# Autodesk Inventor assembly: Tiger
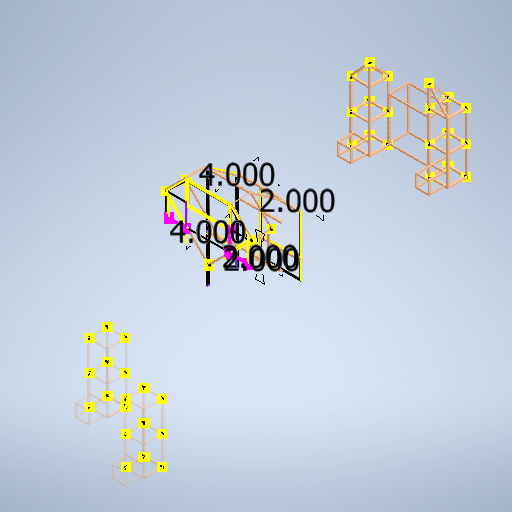
[picture p0: Inventor's stored thumbnail of the model, 512x512]
Saved by Autodesk Inventor 2025 (Build 290162000, 162)
## iProperties
Created: 2024-06-05
Part Number: Tiger
Document SubType Name: Assembly
Designer: Cupri
Mass: 180546 g
Surface Area: 136258 cm^2
Volume: 328266 cm^3
Density: 0.55 g/cm^3
Author: Cupri
## Documents named in this file (26)
- C:\Users\localadmin\Documents\USCTigerBurn24\v2\Tiger.iam
- C:\Users\localadmin\Documents\USCTigerBurn24\Standard Timber\4x4x72.ipt
- C:\Users\localadmin\Documents\USCTigerBurn24\Standard Timber\4x4x40.ipt
- C:\Users\localadmin\Documents\USCTigerBurn24\Standard Timber\2x4x36.ipt
- C:\Users\localadmin\Documents\USCTigerBurn24\Standard Timber\2x4x40.ipt
- C:\Users\localadmin\Documents\USCTigerBurn24\Standard Timber\2x4x24.ipt
- C:\Users\localadmin\Documents\USCTigerBurn24\Standard Timber\2x4x28.ipt
- C:\Users\localadmin\Documents\USCTigerBurn24\Standard Timber\2x4x72 (45 90).ipt
- C:\Users\localadmin\Documents\USCTigerBurn24\Standard Timber\2x4x68 (45 90).ipt
- C:\Users\localadmin\Documents\USCTigerBurn24\Standard Timber\2x4x42.343 (45 90).ipt
- C:\Users\localadmin\Documents\USCTigerBurn24\Standard Timber\2x4x72 (30 90).ipt
- C:\Users\localadmin\Documents\USCTigerBurn24\Standard Timber\2x4x44.ipt
- C:\Users\localadmin\Documents\USCTigerBurn24\Standard Timber\4x4x104.303.ipt
- C:\Users\localadmin\Documents\USCTigerBurn24\Standard Timber\4x4xidkanymore.ipt
- C:\Users\localadmin\Documents\USCTigerBurn24\Standard Timber\4x4x48.ipt
- C:\Users\localadmin\Documents\USCTigerBurn24\Standard Timber\4x4xigiveup.ipt
- C:\Users\localadmin\Documents\USCTigerBurn24\Standard Timber\4x4x96.ipt
- C:\Users\localadmin\Documents\USCTigerBurn24\Standard Timber\2x4x96.ipt
- C:\Users\localadmin\Documents\USCTigerBurn24\Standard Timber\2x4xidk.ipt
- C:\Users\localadmin\Documents\Back right leg.ipt
- C:\Users\localadmin\Documents\USCTigerBurn24\v2\Tiger\AIP\FEA\epzzwi8io.fins
- C:\Users\localadmin\Documents\USCTigerBurn24\v2\Tiger\AIP\FEA\epzzwi8io.fsat
- C:\Users\localadmin\Documents\USCTigerBurn24\v2\Tiger\AIP\FEA\epzzwi8io.ftes
- C:\Users\localadmin\Documents\USCTigerBurn24\v2\Tiger\AIP\FEA\epzzwi8io.fwiz
- C:\Users\localadmin\Documents\USCTigerBurn24\v2\Tiger\AIP\FEA\epzzwi8jk.fmsh
- C:\Users\localadmin\Documents\USCTigerBurn24\v2\Tiger\AIP\FEA\epzzwi8jl.fres
## Components (173 placed, 19 different names)
1. 4x4x104.303:1 — Flush:221, Flush:222
2. 4x4x104.303:2 — Flush:221, Flush:222
3. 4x4xigiveup:1 — Mate:186
4. 4x4xigiveup:2 — Flush:237, Mate:187, Mate:188
5. 4x4x96:1 — Flush:232
6. 4x4x96:2 — Flush:232
7. 4x4x96:3 — Flush:230
8. 4x4x96:4 — Flush:230
9. 4x4x96:5
10. 2x4x96:1 — Mate:186, Flush:237, Mate:187, Mate:188, Mate:191
11. 2x4xidk:1 — Mate:189, Mate:190, Mate:191, Flush:241
12. 2x4xidk:2 — Mate:192, Flush:240, Flush:241
13. Back right leg:1
14. 2x4x96:2 — Mate:260, Mate:261, Mate:262, Mate:263, Mate:264, Flush:347, Mate:286
15. 2x4x96:3 — Mate:265, Mate:266, Mate:283, Mate:284
16. 2x4x44:5 — Mate:260, Mate:261, Mate:262
17. 2x4x44:7 — Mate:263, Mate:264, Mate:265, Mate:266, Mate:285
18. 2x4x96:4 — Mate:277, Mate:278, Mate:279, Mate:280
19. 2x4x96:5 — Mate:275, Mate:281, Mate:282
20. 2x4x44:8 — Mate:274, Mate:276
21. 2x4x44:9
22. 2x4x96:8 — Mate:274, Mate:275, Mate:276, Mate:283
23. 2x4x96:9 — Mate:277, Mate:278, Flush:347, Mate:286
24. 2x4x96:10 — Mate:279, Mate:280, Mate:285, Flush:348
25. 2x4x96:11 — Mate:281, Mate:282, Mate:284, Mate:287
26. 2x4x72 (45 90):1 — Flush:88
27. 2x4x68 (45 90):1 — Flush:44, Flush:88
28. 2x4x72 (45 90):2 — Flush:48, Mate:48, Flush:51, Mate:49
29. 2x4x72 (45 90):3 — Flush:44, Mate:45, Mate:50, Flush:52, Mate:51
30. 2x4x42.343 (45 90):1 — Flush:48
31. 2x4x42.343 (45 90):2 — Mate:45
32. 2x4x72 (30 90):1 — Mate:48, Flush:51, Mate:49, Flush:70, Flush:238, Mate:192, Flush:240
33. 2x4x72 (30 90):2 — Mate:50, Flush:52, Mate:51, Flush:71, Flush:72
34. 2x4x72 (45 90):4 — Mate:61, Flush:61, Flush:62
35. 2x4x68 (45 90):2 — Mate:61, Flush:61, Flush:62
36. 2x4x72 (45 90):5 — Flush:59, Mate:59, Mate:65, Flush:67, Flush:68
37. 2x4x72 (45 90):6 — Flush:63, Flush:64, Mate:68, Flush:73
38. 2x4x42.343 (45 90):3 — Flush:59, Mate:59
39. 2x4x42.343 (45 90):4 — Flush:63
40. 2x4x72 (30 90):3 — Mate:66, Flush:69, Flush:204, Mate:189
41. 2x4x72 (30 90):4 — Flush:64, Mate:67, Mate:69, Flush:239
42. 2x4x44:1 — Mate:67, Flush:71, Flush:72, Flush:239, Mate:190
43. 2x4x44:2 — Mate:65, Flush:67, Flush:68
44. 2x4x44:3 — Mate:66, Flush:69, Flush:70, Flush:204, Flush:238
45. 2x4x44:4 — Mate:68, Flush:73, Mate:69
46. 4x4x72:49
47. 4x4x72:50 — Mate:287, Flush:348
48. 4x4x40:93
49. 4x4x40:94
50. 4x4x40:95
51. 4x4x40:96
52. 4x4x40:97
53. 4x4x40:98
54. 4x4x40:99
55. 4x4x40:100
56. 4x4x72:51
57. 4x4x72:52
58. 2x4x40:5
59. 2x4x36:17
60. 2x4x36:18
61. 2x4x36:19
62. 2x4x36:20
63. 2x4x24:9
64. 2x4x24:10
65. 2x4x28:9
66. 2x4x28:10
67. 4x4x72:53
68. 4x4x72:54
69. 4x4x40:101
70. 4x4x40:102
71. 4x4x40:103
72. 4x4x40:104
73. 4x4x72:55
74. 4x4x72:56
75. 4x4xidkanymore:5
76. 4x4x48:3
77. 4x4xidkanymore:6
78. 4x4x72:57
79. 4x4x72:58
80. 4x4x40:105
81. 4x4x40:106
82. 4x4x40:107
83. 4x4x40:108
84. 4x4x40:109
85. 4x4x40:110
86. 4x4x40:111
87. 4x4x40:112
88. 4x4x72:59
89. 4x4x72:60
90. 2x4x40:6
91. 2x4x36:21
92. 2x4x36:22
93. 2x4x36:23
94. 2x4x36:24
95. 2x4x24:11
96. 2x4x24:12
97. 2x4x28:11
98. 2x4x28:12
99. 4x4x72:61
100. 4x4x72:62
101. 4x4x40:113
102. 4x4x40:114
103. 4x4x40:115
104. 4x4x40:116
105. 4x4x72:63
106. 4x4x72:64
107. 4x4xidkanymore:7
108. 4x4x48:4
109. 4x4xidkanymore:8
110. 4x4x72:65
111. 4x4x72:66
112. 4x4x40:117
113. 4x4x40:118
114. 4x4x40:119
115. 4x4x40:120
116. 4x4x40:121
117. 4x4x40:122
118. 4x4x40:123
119. 4x4x40:124
120. 4x4x72:67
121. 4x4x72:68
122. 4x4x40:125
123. 4x4x40:126
124. 4x4x40:127
125. 2x4x40:7
126. 2x4x36:25
127. 2x4x36:26
128. 2x4x36:27
129. 2x4x36:28
130. 2x4x24:13
131. 2x4x24:14
132. 2x4x28:13
133. 2x4x28:14
134. 4x4x72:69
135. 4x4x72:70
136. 4x4x40:128
137. 4x4x40:129
138. 4x4x40:130
139. 4x4x40:131
140. 4x4x72:71
141. 4x4x72:72
142. 4x4x72:73
143. 4x4x72:74
144. 4x4x40:132
145. 4x4x40:133
146. 4x4x40:134
147. 4x4x40:135
148. 4x4x40:136
149. 4x4x40:137
150. 4x4x40:138
151. 4x4x40:139
152. 4x4x72:75
153. 4x4x72:76
154. 4x4x40:140
155. 4x4x40:141
156. 4x4x40:142
157. 2x4x40:8
158. 2x4x36:29
159. 2x4x36:30
160. 2x4x36:31
161. 2x4x36:32
162. 2x4x24:15
163. 2x4x24:16
164. 2x4x28:15
165. 2x4x28:16
166. 4x4x72:77
167. 4x4x72:78
168. 4x4x40:143
169. 4x4x40:144
170. 4x4x40:145
171. 4x4x40:146
172. 4x4x72:79
173. 4x4x72:80
## Relationships (335: Flush 138, Mate 119, WeldJoint 78)
- Flush:44: 2x4x68 (45 90):1 ↔ 2x4x72 (45 90):3
- Flush:48: 2x4x72 (45 90):2 ↔ 2x4x42.343 (45 90):1
- Mate:45: 2x4x72 (45 90):3 ↔ 2x4x42.343 (45 90):2
- Mate:48: 2x4x72 (45 90):2 ↔ 2x4x72 (30 90):1
- Flush:51: 2x4x72 (45 90):2 ↔ 2x4x72 (30 90):1
- Mate:49: 2x4x72 (45 90):2 ↔ 2x4x72 (30 90):1
- Mate:50: 2x4x72 (45 90):3 ↔ 2x4x72 (30 90):2
- Flush:52: 2x4x72 (45 90):3 ↔ 2x4x72 (30 90):2
- Mate:51: 2x4x72 (45 90):3 ↔ 2x4x72 (30 90):2
- [Flush]: 2x4x68 (45 90):2 ↔ 2x4x72 (45 90):6
- [Flush]: 2x4x72 (45 90):5 ↔ 2x4x42.343 (45 90):3
- [Mate]: 2x4x72 (45 90):6 ↔ 2x4x42.343 (45 90):4
- [Mate]: 2x4x72 (45 90):5 ↔ 2x4x72 (30 90):3
- [Flush]: 2x4x72 (45 90):5 ↔ 2x4x72 (30 90):3
- [Mate]: 2x4x72 (45 90):5 ↔ 2x4x72 (30 90):3
- [Mate]: 2x4x72 (45 90):6 ↔ 2x4x72 (30 90):4
- [Flush]: 2x4x72 (45 90):6 ↔ 2x4x72 (30 90):4
- [Mate]: 2x4x72 (45 90):6 ↔ 2x4x72 (30 90):4
- Flush:59: 2x4x72 (45 90):5 ↔ 2x4x42.343 (45 90):3
- Mate:59: 2x4x72 (45 90):5 ↔ 2x4x42.343 (45 90):3
- Mate:61: 2x4x72 (45 90):4 ↔ 2x4x68 (45 90):2
- Flush:61: 2x4x72 (45 90):4 ↔ 2x4x68 (45 90):2
- Flush:62: 2x4x72 (45 90):4 ↔ 2x4x68 (45 90):2
- Flush:63: 2x4x72 (45 90):6 ↔ 2x4x42.343 (45 90):4
- Flush:64: 2x4x72 (45 90):6 ↔ 2x4x72 (30 90):4
- Mate:65: 2x4x72 (45 90):5 ↔ 2x4x44:2
- Flush:67: 2x4x72 (45 90):5 ↔ 2x4x44:2
- Flush:68: 2x4x72 (45 90):5 ↔ 2x4x44:2
- Mate:66: 2x4x72 (30 90):3 ↔ 2x4x44:3
- Flush:69: 2x4x72 (30 90):3 ↔ 2x4x44:3
- Flush:70: 2x4x72 (30 90):1 ↔ 2x4x44:3
- Mate:67: 2x4x72 (30 90):4 ↔ 2x4x44:1
- Flush:71: 2x4x72 (30 90):2 ↔ 2x4x44:1
- Flush:72: 2x4x72 (30 90):2 ↔ 2x4x44:1
- Mate:68: 2x4x72 (45 90):6 ↔ 2x4x44:4
- Flush:73: 2x4x72 (45 90):6 ↔ 2x4x44:4
- Mate:69: 2x4x72 (30 90):4 ↔ 2x4x44:4
- Flush:88: 2x4x72 (45 90):1 ↔ 2x4x68 (45 90):1
- Flush:204: 2x4x72 (30 90):3 ↔ 2x4x44:3
- Flush:221: 4x4x104.303:1 ↔ 4x4x104.303:2
- Flush:222: 4x4x104.303:1 ↔ 4x4x104.303:2
- Flush:230: 4x4x96:3 ↔ 4x4x96:4
- Flush:232: 4x4x96:1 ↔ 4x4x96:2
- Mate:186: 4x4xigiveup:1 ↔ 2x4x96:1
- Flush:237: 4x4xigiveup:2 ↔ 2x4x96:1
- Mate:187: 4x4xigiveup:2 ↔ 2x4x96:1
- Mate:188: 4x4xigiveup:2 ↔ 2x4x96:1
- Flush:238: 2x4x72 (30 90):1 ↔ 2x4x44:3
- Flush:239: 2x4x72 (30 90):4 ↔ 2x4x44:1
- Mate:189: 2x4xidk:1 ↔ 2x4x72 (30 90):3
- Mate:190: 2x4xidk:1 ↔ 2x4x44:1
- Mate:191: 2x4x96:1 ↔ 2x4xidk:1
- Mate:192: 2x4xidk:2 ↔ 2x4x72 (30 90):1
- Flush:240: 2x4xidk:2 ↔ 2x4x72 (30 90):1
- Flush:241: 2x4xidk:1 ↔ 2x4xidk:2
- [WeldJoint]: 4x4x72:49 ↔ 4x4x40:93
- [WeldJoint]: 4x4x72:50 ↔ 4x4x40:93
- [WeldJoint]: 4x4x72:49 ↔ 4x4x40:94
- [WeldJoint]: 4x4x72:50 ↔ 4x4x40:96
- [WeldJoint]: 4x4x40:94 ↔ 4x4x72:51
- [WeldJoint]: 4x4x40:95 ↔ 4x4x72:51
- [WeldJoint]: 4x4x40:96 ↔ 4x4x72:52
- [WeldJoint]: 4x4x72:50 ↔ 4x4x40:97
- [WeldJoint]: 4x4x40:98 ↔ 4x4x72:51
- [WeldJoint]: 4x4x72:49 ↔ 4x4x40:100
- [WeldJoint]: 4x4x72:49 ↔ 4x4x40:99
- [Mate]: 4x4x72:51 ↔ 2x4x40:5
- [Flush]: 4x4x72:51 ↔ 2x4x40:5
- [Mate] (609.6 mm): 4x4x40:95 ↔ 2x4x40:5
- [Mate] (101.6 mm): 4x4x40:95 ↔ 2x4x36:17
- [Flush]: 4x4x40:95 ↔ 2x4x36:17
- [Mate] (101.6 mm): 4x4x72:52 ↔ 2x4x36:20
- [Flush]: 4x4x40:95 ↔ 2x4x36:20
- [Mate] (101.6 mm): 2x4x40:5 ↔ 2x4x36:18
- [Flush]: 2x4x40:5 ↔ 2x4x36:18
- [Mate]: 2x4x40:5 ↔ 2x4x36:19
- [Flush]: 2x4x40:5 ↔ 2x4x36:19
- [Mate]: 2x4x36:19 ↔ 2x4x36:20
- [WeldJoint]: 2x4x36:17 ↔ 2x4x24:9
- [WeldJoint]: 2x4x36:20 ↔ 2x4x24:10
- [WeldJoint]: 2x4x36:19 ↔ 2x4x28:9
- [WeldJoint]: 2x4x36:20 ↔ 2x4x28:10
- [WeldJoint]: 4x4x72:54 ↔ 4x4x40:101
- [WeldJoint]: 4x4x40:102 ↔ 4x4x72:55
- [WeldJoint]: 4x4x72:53 ↔ 4x4x40:104
- [WeldJoint]: 4x4x72:53 ↔ 4x4x40:103
- [Flush]: 2x4x40:5 ↔ 2x4x36:18
- [Flush]: 2x4x40:5 ↔ 2x4x36:19
- [Flush]: 4x4x40:95 ↔ 2x4x36:17
- [Flush]: 4x4x40:95 ↔ 2x4x36:20
- [Flush] (203.2 mm): 4x4x72:52 ↔ 2x4x36:19
- [Flush] (203.2 mm): 4x4x72:52 ↔ 2x4x36:20
- [Flush]: 2x4x36:17 ↔ 2x4x28:10
- [Mate]: 2x4x36:18 ↔ 2x4x28:9
- [Flush]: 4x4x40:102 ↔ 4x4x72:55
- [Flush]: 4x4x40:102 ↔ 4x4x72:56
- [Mate]: 4x4x40:102 ↔ 4x4x72:56
- [Mate]: 4x4x40:101 ↔ 4x4x72:56
- [Flush]: 4x4x40:101 ↔ 4x4x72:56
- [Flush]: 4x4x72:54 ↔ 4x4x40:101
- [Mate]: 4x4x72:54 ↔ 4x4x40:101
- [Flush]: 4x4x72:53 ↔ 4x4x40:104
- [Flush]: 4x4x72:53 ↔ 4x4x40:103
- [Mate]: 4x4x72:51 ↔ 2x4x40:5
- [Mate]: 2x4x36:18 ↔ 2x4x24:9
- [Flush]: 4x4x72:52 ↔ 4x4x72:56
- [Flush]: 4x4x72:50 ↔ 4x4x40:97
- [Mate]: 4x4x72:50 ↔ 4x4x72:54
- [Flush]: 4x4x72:50 ↔ 4x4x72:54
- [Flush]: 4x4x72:49 ↔ 4x4x72:53
- [Mate]: 4x4x72:49 ↔ 4x4x72:53
- [Flush]: 4x4x72:49 ↔ 4x4x72:53
- [Mate]: 4x4x72:51 ↔ 4x4x72:55
- [Flush]: 4x4x72:51 ↔ 4x4x72:55
- [Flush]: 4x4x72:51 ↔ 4x4x72:55
- [Mate]: 2x4x36:17 ↔ 2x4x28:10
- [Flush]: 2x4x36:18 ↔ 2x4x24:9
- [Flush]: 2x4x36:18 ↔ 2x4x28:9
- [Flush]: 4x4x72:54 ↔ 4x4x40:103
- [Flush]: 4x4x40:101 ↔ 4x4x40:104
- [Flush]: 4x4x72:53 ↔ 4x4x40:103
- [Flush]: 4x4x40:102 ↔ 4x4x72:55
- [Flush]: 4x4x40:102 ↔ 4x4x72:56
- [WeldJoint]: 4x4x72:54 ↔ 4x4xidkanymore:5
- [Flush]: 4x4x72:54 ↔ 4x4xidkanymore:5
- [Flush]: 4x4x40:101 ↔ 4x4xidkanymore:5
- [Mate]: 4x4x72:56 ↔ 4x4x48:3
- [Flush]: 4x4x72:56 ↔ 4x4x48:3
- [Flush]: 4x4x72:56 ↔ 4x4x48:3
- [Mate]: 4x4x48:3 ↔ 4x4xidkanymore:6
- [Flush]: 4x4x48:3 ↔ 4x4xidkanymore:6
- [Mate]: 4x4x40:102 ↔ 4x4xidkanymore:6
- [WeldJoint]: 4x4x72:57 ↔ 4x4x40:105
- [WeldJoint]: 4x4x72:58 ↔ 4x4x40:105
- [WeldJoint]: 4x4x72:57 ↔ 4x4x40:106
- [WeldJoint]: 4x4x72:58 ↔ 4x4x40:108
- [WeldJoint]: 4x4x40:106 ↔ 4x4x72:59
- [WeldJoint]: 4x4x40:107 ↔ 4x4x72:59
- [WeldJoint]: 4x4x40:108 ↔ 4x4x72:60
- [WeldJoint]: 4x4x72:58 ↔ 4x4x40:109
- [WeldJoint]: 4x4x40:110 ↔ 4x4x72:59
- [WeldJoint]: 4x4x72:57 ↔ 4x4x40:112
- [WeldJoint]: 4x4x72:57 ↔ 4x4x40:111
- [Mate]: 4x4x72:59 ↔ 2x4x40:6
- [Flush]: 4x4x72:59 ↔ 2x4x40:6
- [Mate] (609.6 mm): 4x4x40:107 ↔ 2x4x40:6
- [Mate] (101.6 mm): 4x4x40:107 ↔ 2x4x36:21
- [Flush]: 4x4x40:107 ↔ 2x4x36:21
- [Mate] (101.6 mm): 4x4x72:60 ↔ 2x4x36:24
- [Flush]: 4x4x40:107 ↔ 2x4x36:24
- [Mate] (101.6 mm): 2x4x40:6 ↔ 2x4x36:22
- [Flush]: 2x4x40:6 ↔ 2x4x36:22
- [Mate]: 2x4x40:6 ↔ 2x4x36:23
- [Flush]: 2x4x40:6 ↔ 2x4x36:23
- [Mate]: 2x4x36:23 ↔ 2x4x36:24
- [WeldJoint]: 2x4x36:21 ↔ 2x4x24:11
- [WeldJoint]: 2x4x36:24 ↔ 2x4x24:12
- [WeldJoint]: 2x4x36:23 ↔ 2x4x28:11
- [WeldJoint]: 2x4x36:24 ↔ 2x4x28:12
- [WeldJoint]: 4x4x72:62 ↔ 4x4x40:113
- [WeldJoint]: 4x4x40:114 ↔ 4x4x72:63
- [WeldJoint]: 4x4x72:61 ↔ 4x4x40:116
- [WeldJoint]: 4x4x72:61 ↔ 4x4x40:115
- [Flush]: 2x4x40:6 ↔ 2x4x36:22
- [Flush]: 2x4x40:6 ↔ 2x4x36:23
- [Flush]: 4x4x40:107 ↔ 2x4x36:21
- [Flush]: 4x4x40:107 ↔ 2x4x36:24
- [Flush] (203.2 mm): 4x4x72:60 ↔ 2x4x36:23
- [Flush] (203.2 mm): 4x4x72:60 ↔ 2x4x36:24
- [Flush]: 2x4x36:21 ↔ 2x4x28:12
- [Mate]: 2x4x36:22 ↔ 2x4x28:11
- [Flush]: 4x4x40:114 ↔ 4x4x72:63
- [Flush]: 4x4x40:114 ↔ 4x4x72:64
- [Mate]: 4x4x40:114 ↔ 4x4x72:64
- [Mate]: 4x4x40:113 ↔ 4x4x72:64
- [Flush]: 4x4x40:113 ↔ 4x4x72:64
- [Flush]: 4x4x72:62 ↔ 4x4x40:113
- [Mate]: 4x4x72:62 ↔ 4x4x40:113
- [Flush]: 4x4x72:61 ↔ 4x4x40:116
- [Flush]: 4x4x72:61 ↔ 4x4x40:115
- [Mate]: 4x4x72:59 ↔ 2x4x40:6
- [Mate]: 2x4x36:22 ↔ 2x4x24:11
- [Flush]: 4x4x72:60 ↔ 4x4x72:64
- [Flush]: 4x4x72:58 ↔ 4x4x40:109
- [Mate]: 4x4x72:58 ↔ 4x4x72:62
- [Flush]: 4x4x72:58 ↔ 4x4x72:62
- [Flush]: 4x4x72:57 ↔ 4x4x72:61
- [Mate]: 4x4x72:57 ↔ 4x4x72:61
- [Flush]: 4x4x72:57 ↔ 4x4x72:61
- [Mate]: 4x4x72:59 ↔ 4x4x72:63
- [Flush]: 4x4x72:59 ↔ 4x4x72:63
- [Flush]: 4x4x72:59 ↔ 4x4x72:63
- [Mate]: 2x4x36:21 ↔ 2x4x28:12
- [Flush]: 2x4x36:22 ↔ 2x4x24:11
- [Flush]: 2x4x36:22 ↔ 2x4x28:11
- [WeldJoint]: 4x4x72:61 ↔ 4x4xidkanymore:7
- [Flush]: 4x4x72:61 ↔ 4x4xidkanymore:7
- [Mate]: 4x4x72:63 ↔ 4x4x48:4
- [Flush]: 4x4x72:63 ↔ 4x4x48:4
- [Flush]: 4x4x72:63 ↔ 4x4x48:4
- [Mate]: 4x4x72:64 ↔ 4x4xidkanymore:8
- [Mate]: 4x4x48:4 ↔ 4x4xidkanymore:8
- [Flush]: 4x4x48:4 ↔ 4x4xidkanymore:8
- [WeldJoint]: 4x4x72:65 ↔ 4x4x40:117
- [WeldJoint]: 4x4x72:66 ↔ 4x4x40:117
- [WeldJoint]: 4x4x72:65 ↔ 4x4x40:118
- [WeldJoint]: 4x4x72:66 ↔ 4x4x40:120
- [WeldJoint]: 4x4x40:118 ↔ 4x4x72:67
- [WeldJoint]: 4x4x40:119 ↔ 4x4x72:67
- [WeldJoint]: 4x4x40:120 ↔ 4x4x72:68
- [WeldJoint]: 4x4x72:66 ↔ 4x4x40:121
- [WeldJoint]: 4x4x40:122 ↔ 4x4x72:67
- [WeldJoint]: 4x4x72:65 ↔ 4x4x40:124
- [WeldJoint]: 4x4x72:65 ↔ 4x4x40:123
- [Mate]: 4x4x72:67 ↔ 2x4x40:7
- [Flush]: 4x4x72:67 ↔ 2x4x40:7
- [Mate] (609.6 mm): 4x4x40:119 ↔ 2x4x40:7
- [Mate] (101.6 mm): 4x4x40:119 ↔ 2x4x36:25
- [Flush]: 4x4x40:119 ↔ 2x4x36:25
- [Mate] (101.6 mm): 4x4x72:68 ↔ 2x4x36:28
- [Flush]: 4x4x40:119 ↔ 2x4x36:28
- [Mate] (101.6 mm): 2x4x40:7 ↔ 2x4x36:26
- [Flush]: 2x4x40:7 ↔ 2x4x36:26
- [Mate]: 2x4x40:7 ↔ 2x4x36:27
- [Flush]: 2x4x40:7 ↔ 2x4x36:27
- [Mate]: 2x4x36:27 ↔ 2x4x36:28
- [WeldJoint]: 2x4x36:25 ↔ 2x4x24:13
- [WeldJoint]: 2x4x36:28 ↔ 2x4x24:14
- [WeldJoint]: 2x4x36:27 ↔ 2x4x28:13
- [WeldJoint]: 2x4x36:28 ↔ 2x4x28:14
- [WeldJoint]: 4x4x72:70 ↔ 4x4x40:128
- [WeldJoint]: 4x4x40:129 ↔ 4x4x72:71
- [WeldJoint]: 4x4x72:69 ↔ 4x4x40:131
- [WeldJoint]: 4x4x72:69 ↔ 4x4x40:130
- [Flush]: 2x4x40:7 ↔ 2x4x36:26
- [Flush]: 2x4x40:7 ↔ 2x4x36:27
- [Flush]: 4x4x40:119 ↔ 2x4x36:25
- [Flush]: 4x4x40:119 ↔ 2x4x36:28
- [Flush] (203.2 mm): 4x4x72:68 ↔ 2x4x36:27
- [Flush] (203.2 mm): 4x4x72:68 ↔ 2x4x36:28
- [Flush]: 2x4x36:25 ↔ 2x4x28:14
- [Mate]: 2x4x36:26 ↔ 2x4x28:13
- [Flush]: 4x4x40:129 ↔ 4x4x72:71
- [Flush]: 4x4x40:129 ↔ 4x4x72:72
- [Mate]: 4x4x40:129 ↔ 4x4x72:72
- [Mate]: 4x4x40:128 ↔ 4x4x72:72
- [Flush]: 4x4x40:128 ↔ 4x4x72:72
- [Flush]: 4x4x72:70 ↔ 4x4x40:128
- [Mate]: 4x4x72:70 ↔ 4x4x40:128
- [Flush]: 4x4x72:69 ↔ 4x4x40:131
- [Flush]: 4x4x72:69 ↔ 4x4x40:130
- [Mate]: 4x4x72:67 ↔ 2x4x40:7
- [Mate]: 2x4x36:26 ↔ 2x4x24:13
- [Flush]: 4x4x72:68 ↔ 4x4x72:72
- [Flush]: 4x4x72:68 ↔ 4x4x72:72
- [WeldJoint]: 4x4x72:73 ↔ 4x4x40:132
- [WeldJoint]: 4x4x72:74 ↔ 4x4x40:132
- [WeldJoint]: 4x4x72:73 ↔ 4x4x40:133
- [WeldJoint]: 4x4x72:74 ↔ 4x4x40:135
- [WeldJoint]: 4x4x40:133 ↔ 4x4x72:75
- [WeldJoint]: 4x4x40:134 ↔ 4x4x72:75
- [WeldJoint]: 4x4x40:135 ↔ 4x4x72:76
- [WeldJoint]: 4x4x72:74 ↔ 4x4x40:136
- [WeldJoint]: 4x4x40:137 ↔ 4x4x72:75
- [WeldJoint]: 4x4x72:73 ↔ 4x4x40:139
- [WeldJoint]: 4x4x72:73 ↔ 4x4x40:138
- [Mate]: 4x4x72:75 ↔ 2x4x40:8
- [Flush]: 4x4x72:75 ↔ 2x4x40:8
- [Mate] (609.6 mm): 4x4x40:134 ↔ 2x4x40:8
- [Mate] (101.6 mm): 4x4x40:134 ↔ 2x4x36:29
- [Flush]: 4x4x40:134 ↔ 2x4x36:29
- [Mate] (101.6 mm): 4x4x72:76 ↔ 2x4x36:32
- [Flush]: 4x4x40:134 ↔ 2x4x36:32
- [Mate]: 2x4x40:8 ↔ 2x4x36:31
- [Flush]: 2x4x40:8 ↔ 2x4x36:31
- [Mate]: 2x4x36:31 ↔ 2x4x36:32
- [WeldJoint]: 2x4x36:29 ↔ 2x4x24:15
- [WeldJoint]: 2x4x36:32 ↔ 2x4x24:16
- [WeldJoint]: 2x4x36:31 ↔ 2x4x28:15
- [WeldJoint]: 2x4x36:32 ↔ 2x4x28:16
- [WeldJoint]: 4x4x72:78 ↔ 4x4x40:143
- [WeldJoint]: 4x4x40:144 ↔ 4x4x72:79
- [WeldJoint]: 4x4x72:77 ↔ 4x4x40:146
- [WeldJoint]: 4x4x72:77 ↔ 4x4x40:145
- [Flush]: 2x4x40:8 ↔ 2x4x36:31
- [Flush]: 4x4x40:134 ↔ 2x4x36:29
- [Flush]: 4x4x40:134 ↔ 2x4x36:32
- [Flush] (203.2 mm): 4x4x72:76 ↔ 2x4x36:31
- [Flush] (203.2 mm): 4x4x72:76 ↔ 2x4x36:32
- [Flush]: 2x4x36:29 ↔ 2x4x28:16
- [Flush]: 2x4x36:30 ↔ 2x4x28:15
- [Mate]: 2x4x36:30 ↔ 2x4x28:15
- [Flush]: 4x4x40:144 ↔ 4x4x72:79
- [Flush]: 4x4x40:144 ↔ 4x4x72:80
- [Mate]: 4x4x40:144 ↔ 4x4x72:79
- [Mate]: 4x4x40:146 ↔ 4x4x72:79
- [Mate]: 4x4x72:74 ↔ 4x4x72:78
- [Mate]: 4x4x72:75 ↔ 2x4x40:8
- [Mate]: 2x4x40:8 ↔ 2x4x24:15
- [Flush]: 2x4x36:31 ↔ 2x4x24:16
- [Flush]: 2x4x36:31 ↔ 2x4x24:16
- [Mate]: 2x4x40:8 ↔ 2x4x36:30
- [Flush]: 2x4x36:30 ↔ 2x4x28:15
- [Flush]: 2x4x36:30 ↔ 2x4x28:15
- [Mate]: 4x4x72:78 ↔ 4x4x40:145
- Mate:260: 2x4x96:2 ↔ 2x4x44:5
- Mate:261: 2x4x96:2 ↔ 2x4x44:5
- Mate:262: 2x4x96:2 ↔ 2x4x44:5
- Mate:263: 2x4x96:2 ↔ 2x4x44:7
- Mate:264: 2x4x96:2 ↔ 2x4x44:7
- Mate:265: 2x4x96:3 ↔ 2x4x44:7
- Mate:266: 2x4x96:3 ↔ 2x4x44:7
- [Mate]: 2x4x96:4 ↔ 2x4x44:8
- [Mate]: 2x4x96:4 ↔ 2x4x44:8
- [Mate]: 2x4x96:4 ↔ 2x4x44:8
- [Mate]: 2x4x96:4 ↔ 2x4x44:9
- [Mate]: 2x4x96:4 ↔ 2x4x44:9
- [Mate]: 2x4x96:5 ↔ 2x4x44:9
- [Mate]: 2x4x96:5 ↔ 2x4x44:9
- Mate:274: 2x4x44:8 ↔ 2x4x96:8
- Mate:275: 2x4x96:5 ↔ 2x4x96:8
- Mate:276: 2x4x44:8 ↔ 2x4x96:8
- Mate:277: 2x4x96:4 ↔ 2x4x96:9
- Mate:278: 2x4x96:4 ↔ 2x4x96:9
- Mate:279: 2x4x96:4 ↔ 2x4x96:10
- Mate:280: 2x4x96:4 ↔ 2x4x96:10
- Mate:281: 2x4x96:5 ↔ 2x4x96:11
- Mate:282: 2x4x96:5 ↔ 2x4x96:11
- Mate:283: 2x4x96:3 ↔ 2x4x96:8
- Flush:347: 2x4x96:2 ↔ 2x4x96:9
- Mate:284: 2x4x96:3 ↔ 2x4x96:11
- Mate:285: 2x4x44:7 ↔ 2x4x96:10
- Mate:286: 2x4x96:2 ↔ 2x4x96:9
- Mate:287: 2x4x96:11 ↔ 4x4x72:50
- Flush:348: 2x4x96:10 ↔ 4x4x72:50
## Named parameters: sa_0 = 22241.1, d253_d234 = 0 mm, d254_d240 = 0 mm, d255_d242 = 0 mm, d256_d247 = 0 mm, d257_d248 = 0 mm, d258_d249 = 0 mm, d259_d250 = 0 mm, d260_d251 = 0 mm, d261_d252 = 0 mm, sa_1 = 980.999, d679_d599 = 0 mm, d680_d600 = 0 mm, d681_d601 = 0 mm, d682_d602 = 0 mm, d683_d603 = 0 mm, d684_d605 = 0 mm, d685_d608 = 0 mm, d686_d609 = 0 mm, d687_d610 = 0 mm, d688_d611 = 0 mm, d689_d612 = 0 mm, d690_d619 = 0 mm, d691_d620 = 0 mm, d692_d621 = 0 mm, d693_d561_d429_d35 = 0 mm, d694_d562_d430_d36 = 0 mm, d695_d563_d431_d37 = 0 mm, d696_d564_d432_d38 = 0 mm, d697_d565_d505 = 0 mm, d698_d566_d506 = 0 mm, d699_d567_d507 = 0 mm, d700_d568_d508 = 0 mm, d701_d569_d509 = 0 mm, d702_d570_d512 = 0 mm, d703_d571_d513 = 0 mm, d704_d572_d514 = 0 mm, d705_d573_d498 = 0 mm, d706_d574_d501 = 0 mm, d707_d575_d502 = 0 mm, d708_d576_d503 = 0 mm, d709_d577_d504 = 0 mm, d710_d515_d433_d39 = 0 mm, d711_d516_d434_d29 = 0 mm, d712_d517_d435_d30 = 0 mm, d713_d518_d436_d326 = 0 mm, d714_d519_d437_d327 = 0 mm, d715_d520_d438_d314 = 0 mm, d716_d521_d439_d315 = 0 mm, d717_d522_d440_d316 = 0 mm, d718_d523_d441_d317 = 0 mm, d719_d524_d442_d305 = 0 mm, d720_d525_d443_d306 = 0 mm, d721_d526_d444_d311 = 0 mm, d722_d527_d445_d312 = 0 mm, d723_d528_d446_d313 = 0 mm, d724_d529_d396_d137_d48_d37 = 0 mm, d725_d530_d397_d138_d49_d38 = 0 mm, d726_d531_d398_d139_d50_d39 = 0 mm, d727_d532_d399_d143 = 0 mm, d728_d533_d400_d144 = 0 mm, d729_d534_d401_d145 = 0 mm, d730_d535_d402_d146 = 0 mm, d731_d536_d403_d147 = 203.2 mm, d732_d537_d404_d148 = 203.2 mm, d733_d538_d405_d149 = 0 mm, d734_d539_d406_d150 = 0 mm, d735_d540_d407_d61 = 0 mm, d736_d541_d408_d62 = 0 mm, d737_d542_d409_d63 = 609.6 mm, d738_d543_d410_d68 = 101.6 mm, d739_d544_d411_d69 = 0 mm, d740_d545_d412_d70 = 101.6 mm, d741_d546_d413_d71 = 0 mm, d742_d547_d414_d72 = 101.6 mm, d743_d548_d415_d73 = 0 mm, d744_d549_d416_d74 = 0 mm, d745_d550_d417_d75 = 0 mm, d746_d551_d418_d76 = 0 mm, d747_d552_d419_d77 = 0 mm, d748_d553_d420_d78 = 0 mm, d749_d554_d421_d79 = 0 mm, d750_d555_d422_d80 = 0 mm, d751_d556_d423_d136_d47_d36 = 0 mm, d752_d557_d425_d31 = 0 mm, d753_d558_d426_d32 = 0 mm, d754_d559_d427_d33 = 0 mm, d755_d560_d428_d34 = 0 mm, d756_d606 = 0 mm, d757_d607 = 0 mm, d758_d613 = 0 mm, d759_d614 = 0 mm, d760_d615 = 0 mm, d761_d616 = 0 mm, d762_d617 = 0 mm, d763_d618 = 0 mm, d764_d502 = 0 mm, d765_d503 = 0 mm, d766_d504 = 0 mm, d767_d505 = 0 mm, d768_d506 = 0 mm, d769_d507 = 0 mm, d770_d508 = 0 mm, d771_d509 = 0 mm, d772_d512 = 0 mm, d773_d513 = 0 mm, d774_d514 = 0 mm, d775_d434_d29 = 0 mm, d776_d435_d30 = 0 mm, d777_d436_d326 = 0 mm, d778_d437_d327 = 0 mm, d779_d438_d314 = 0 mm, d780_d439_d315 = 0 mm, d781_d440_d316 = 0 mm, d782_d441_d317 = 0 mm, d783_d442_d305 = 0 mm, d784_d443_d306 = 0 mm, d785_d444_d311 = 0 mm, d786_d445_d312 = 0 mm, d787_d446_d313 = 0 mm, d788_d498 = 0 mm, d789_d501 = 0 mm, d790_d396_d137_d48_d37 = 0 mm, d791_d397_d138_d49_d38 = 0 mm, d792_d398_d139_d50_d39 = 0 mm, d793_d399_d143 = 0 mm, d794_d400_d144 = 0 mm, d795_d401_d145 = 0 mm, d796_d402_d146 = 0 mm, d797_d403_d147 = 203.2 mm, d798_d404_d148 = 203.2 mm, d799_d405_d149 = 0 mm, d800_d406_d150 = 0 mm, d801_d407_d61 = 0 mm, d802_d408_d62 = 0 mm, d803_d409_d63 = 609.6 mm, d804_d410_d68 = 101.6 mm, d805_d411_d69 = 0 mm, d806_d412_d70 = 101.6 mm, d807_d413_d71 = 0 mm, d808_d414_d72 = 101.6 mm, d809_d415_d73 = 0 mm, d810_d416_d74 = 0 mm, d811_d417_d75 = 0 mm, d812_d418_d76 = 0 mm, d813_d419_d77 = 0 mm, d814_d420_d78 = 0 mm, d815_d421_d79 = 0 mm, d816_d422_d80 = 0 mm, d817_d423_d136_d47_d36 = 0 mm, d818_d425_d31 = 0 mm, d819_d426_d32 = 0 mm, d820_d427_d33 = 0 mm, d821_d428_d34 = 0 mm, d822_d429_d35 = 0 mm, d823_d430_d36 = 0 mm, d824_d431_d37 = 0 mm, d825_d432_d38 = 0 mm, d826_d433_d39 = 0 mm, d827_d499 = 0 mm, d828_d500 = 0 mm, d829_d326 = 0 mm, d830_d327 = 0 mm, d831_d305 = 0 mm, d832_d306 = 0 mm, d833_d311 = 0 mm, d834_d312 = 0 mm, d835_d313 = 0 mm, d836_d314 = 0 mm, d837_d315 = 0 mm, d838_d316 = 0 mm, d839_d317 = 0 mm, d840_d143 = 0 mm, d841_d144 = 0 mm, d842_d145 = 0 mm, d843_d146 = 0 mm, d844_d147 = 203.2 mm, d845_d148 = 203.2 mm, d846_d149 = 0 mm, d847_d150 = 0 mm, d848_d61 = 0 mm, d849_d62 = 0 mm, d850_d63 = 609.6 mm, d851_d68 = 101.6 mm, d852_d69 = 0 mm, d853_d70 = 101.6 mm, d854_d71 = 0 mm, d855_d72 = 101.6 mm, d856_d73 = 0 mm, d857_d74 = 0 mm, d858_d75 = 0 mm, d859_d76 = 0 mm, d860_d77 = 0 mm, d861_d78 = 0 mm, d862_d79 = 0 mm, d863_d80 = 0 mm, d864_d136_d47_d36 = 0 mm, d865_d137_d48_d37 = 0 mm, d866_d138_d49_d38 = 0 mm, d867_d139_d50_d39 = 0 mm, d868_d31 = 0 mm, d869_d32 = 0 mm, d870_d33 = 0 mm, d871_d34 = 0 mm, d872_d35 = 0 mm, d873_d36 = 0 mm, d874_d37 = 0 mm, d875_d38 = 0 mm, d876_d39 = 0 mm, d877_d29 = 0 mm, d878_d30 = 0 mm, d879_d626 = 0 mm, d880_d319 = 0 mm, d881_d320 = 0 mm, d882_d321 = 0 mm, d883_d322 = 0 mm, d884_d323 = 0 mm, d885_d324 = 0 mm, d886_d325 = 0 mm, d887_d299 = 0 mm, d888_d301 = 0 mm, d889_d309 = 0 mm, d890_d310 = 0 mm, d891_d318 = 0 mm, d892_d245 = 0 mm, d893_d246 = 0 mm, d894_d154_d144 = 0 mm, d895_d155_d145 = 0 mm, d896_d156_d146 = 0 mm, d897_d157_d147 = 203.2 mm, d898_d158_d148 = 203.2 mm, d899_d159_d149 = 0 mm, d900_d168_d136_d47_d36 = 0 mm, d901_d169_d137_d48_d37 = 0 mm, d902_d170_d138_d49_d38 = 0 mm, d903_d171_d139_d50_d39 = 0 mm, d904_d173_d61 = 0 mm, d905_d174_d62 = 0 mm, d906_d175_d63 = 609.6 mm, d907_d176_d68 = 101.6 mm, d908_d177_d69 = 0 mm, d909_d178_d70 = 101.6 mm, d910_d179_d71 = 0 mm, d911_d182_d74 = 0 mm, d912_d183_d75 = 0 mm, d913_d184_d76 = 0 mm, d914_d185_d77 = 0 mm, d915_d186_d78 = 0 mm, d916_d187_d79 = 0 mm, d917_d188_d80 = 0 mm, d918_d190_d31 = 0 mm, d919_d191_d32 = 0 mm, d920_d192_d33 = 0 mm, d921_d193_d34 = 0 mm, d922_d194_d35 = 0 mm, d923_d195_d36 = 0 mm, d924_d196_d37 = 0 mm, d925_d197_d38 = 0 mm, d926_d198_d39 = 0 mm, d927_d210_d29 = 0 mm, d928_d211_d30 = 0 mm, d936_d929 = 0 mm, d937_d933 = 0 mm, d938_d934 = 0 mm, d939_d935 = 0 mm, d940_d930 = 0 mm, d941_d931 = 0 mm, d942_d932 = 0 mm
note: some values were not read from the file. Shown as the stored number, unit unknown: "sa_0", "sa_1".
